# Autodesk Inventor assembly: Synchronous Belts Transmission
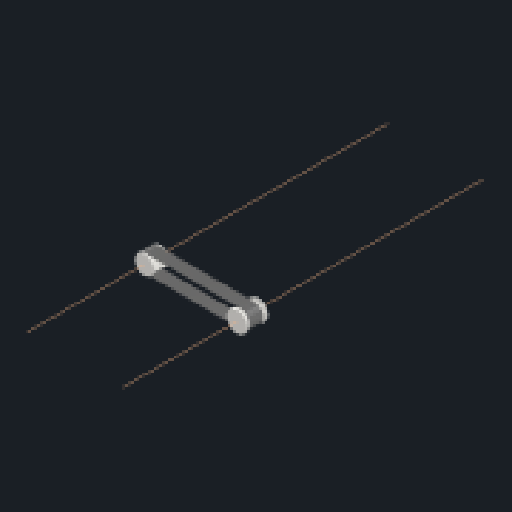
[picture p0: Inventor's stored thumbnail of the model, 512x512]
Saved by Autodesk Inventor 2023.1 (Build 271208000, 208)
## iProperties
ClientObjectVersion: 1
Created: 2023-06-03
Part Number: Synchronous Belts Transmission
Document SubType Name: Assembly
Designer: Jarrett
Author: Jarrett
## Documents named in this file (6)
- C:\Users\Jarrett\Desktop\Projects\BehrendURCMechanical\CAD\Science\Capper Assembly\Design Accelerator\Synchronous Belts Transmission1.iam
- C:\Users\Jarrett\Desktop\Projects\BehrendURCMechanical\CAD\Science\Capper Assembly\Design Accelerator\Synchronous Belt1.ipt
- C:\Users\Jarrett\Desktop\Projects\BehrendURCMechanical\CAD\Science\Capper Assembly\Design Accelerator\Synchronous Pulley11.ipt
- C:\Users\Jarrett\Desktop\Projects\BehrendURCMechanical\CAD\Science\Capper Assembly\Design Accelerator\Synchronous Pulley21.ipt
- C:\Users\Jarrett\Desktop\Projects\BehrendURCMechanical\CAD\Science\Capper Assembly\Design Accelerator\Flat Pulley11.ipt
- C:\Users\Jarrett\Desktop\Projects\BehrendURCMechanical\CAD\Science\Capper Assembly\Design Accelerator\Synchronous Pulley31.ipt
## Components (5 placed, 5 different names)
1. Synchronous Belt:1 — Flush:1, Mate:1, Mate:2, Flush:2, Mate:3, Mate:4, Flush:3, Mate:5, Mate:6, Flush:4, Mate:7
2. Synchronous Pulley1:1 — Flush:1, Mate:1, Mate:2, Rotation:1, Rotation:2, Rotation:3
3. Synchronous Pulley2:1 — Flush:3, Mate:5, Rotation:2, Mate:6
4. Flat Pulley1:1 — Flush:4, Mate:7, Rotation:3
5. Synchronous Pulley3:1 — Flush:2, Mate:3, Rotation:1, Mate:4
## Relationships (14: Mate 7, Flush 4, RelateRotation 3)
- Flush:1: Synchronous Belt:1 ↔ Synchronous Pulley1:1
- Mate:1: Synchronous Belt:1 ↔ Synchronous Pulley1:1
- Mate:2: Synchronous Belt:1 ↔ Synchronous Pulley1:1
- Flush:2: Synchronous Belt:1 ↔ Synchronous Pulley3:1
- Mate:3: Synchronous Belt:1 ↔ Synchronous Pulley3:1
- Rotation:1 [RelateRotation] (0.9259 ul): Synchronous Pulley1:1 ↔ Synchronous Pulley3:1
- Mate:4: Synchronous Belt:1 ↔ Synchronous Pulley3:1
- Flush:3: Synchronous Belt:1 ↔ Synchronous Pulley2:1
- Mate:5: Synchronous Belt:1 ↔ Synchronous Pulley2:1
- Rotation:2 [RelateRotation] (1 ul): Synchronous Pulley1:1 ↔ Synchronous Pulley2:1
- Mate:6: Synchronous Belt:1 ↔ Synchronous Pulley2:1
- Flush:4: Synchronous Belt:1 ↔ Flat Pulley1:1
- Mate:7: Synchronous Belt:1 ↔ Flat Pulley1:1
- Rotation:3 [RelateRotation] (0.8657 ul): Synchronous Pulley1:1 ↔ Flat Pulley1:1
